# Autodesk Inventor assembly: Flexipod2.0
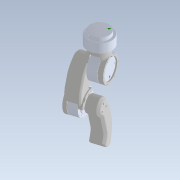
[picture p0: Inventor's stored thumbnail of the model, 180x180]
Saved by Autodesk Inventor 2020 (Build 240168000, 168)
## iProperties
Created: 2020-12-23
Part Number: Flexipod2.0
Document SubType Name: Assembly
Designer: DELL
Author: DELL
## Documents named in this file (6)
- F:\SoftRobot2.0\Flexipod2.0\robot_2020_12_23\Flexipod2.0.iam
- F:\SoftRobot2.0\Flexipod2.0\RMD_X6_stator.ipt
- F:\SoftRobot2.0\Flexipod2.0\RMD_X6_rotor.ipt
- F:\SoftRobot2.0\Flexipod2.0\robot_2020_12_23\hip_link.ipt
- F:\SoftRobot2.0\Flexipod2.0\robot_2020_12_23\thigh_link.ipt
- F:\SoftRobot2.0\Flexipod2.0\robot_2020_12_23\shank_link.ipt
## Components (9 placed, 5 different names)
1. RMD_X6_stator:1 — Mate:1, Flush:1, Mate:14, Mate:15, Mate:16, Mate:17
2. RMD_X6_rotor:1 — Mate:1, Flush:1, Mate:18, Mate:19
3. RMD_X6_stator:2 — Mate:8, Mate:9, Mate:10, Mate:11
4. RMD_X6_rotor:2 — Mate:12, Mate:13
5. RMD_X6_stator:3 — Mate:4, Mate:5
6. RMD_X6_rotor:3 — Mate:6, Mate:7
7. hip_link:1 — Mate:5, Mate:6, Mate:7, Mate:8, Mate:9, Mate:10
8. thigh_link:1 — Mate:11, Mate:12, Mate:13, Mate:14, Mate:15, Mate:16
9. shank_link:1 — Mate:17, Mate:18, Mate:19
## Relationships (22: Mate 19, Flush 3)
- Mate:1: RMD_X6_stator:1 ↔ RMD_X6_rotor:1
- Flush:1 (-3 mm): RMD_X6_stator:1 ↔ RMD_X6_rotor:1
- [Mate]: RMD_X6_stator:2 ↔ RMD_X6_rotor:2
- [Flush] (-3 mm): RMD_X6_stator:2 ↔ RMD_X6_rotor:2
- [Mate]: RMD_X6_stator:3 ↔ RMD_X6_rotor:3
- [Flush] (-3 mm): RMD_X6_stator:3 ↔ RMD_X6_rotor:3
- Mate:4: RMD_X6_stator:3
- Mate:5: RMD_X6_stator:3 ↔ hip_link:1
- Mate:6: RMD_X6_rotor:3 ↔ hip_link:1
- Mate:7: RMD_X6_rotor:3 ↔ hip_link:1
- Mate:8: RMD_X6_stator:2 ↔ hip_link:1
- Mate:9: RMD_X6_stator:2 ↔ hip_link:1
- Mate:10: RMD_X6_stator:2 ↔ hip_link:1
- Mate:11: RMD_X6_stator:2 ↔ thigh_link:1
- Mate:12: RMD_X6_rotor:2 ↔ thigh_link:1
- Mate:13: RMD_X6_rotor:2 ↔ thigh_link:1
- Mate:14: RMD_X6_stator:1 ↔ thigh_link:1
- Mate:15: RMD_X6_stator:1 ↔ thigh_link:1
- Mate:16: RMD_X6_stator:1 ↔ thigh_link:1
- Mate:17: RMD_X6_stator:1 ↔ shank_link:1
- Mate:18: RMD_X6_rotor:1 ↔ shank_link:1
- Mate:19: RMD_X6_rotor:1 ↔ shank_link:1
## Named parameters: d2_d0 = 0 mm, d3_d1 = -3 mm, d4_d0 = 0 mm, d5_d1 = -3 mm
